# Autodesk Inventor assembly: arm_fin1
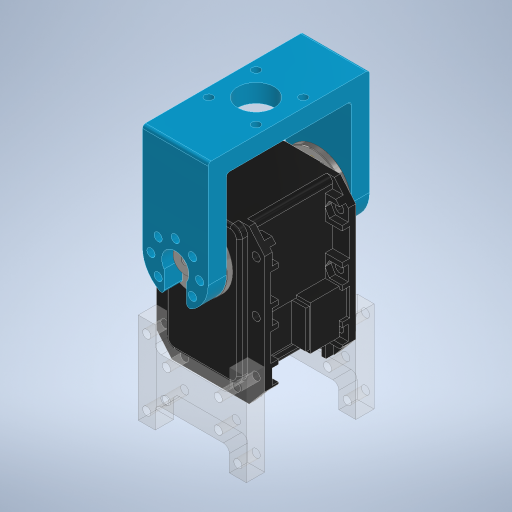
[picture p0: Inventor's stored thumbnail of the model, 512x512]
Saved by Autodesk Inventor 2024 (Build 280153000, 153)
## iProperties
Created: 2024-09-14
Part Number: arm_fin1
Document SubType Name: Assembly
Designer: jmha0
Author: jmha0
## Documents named in this file (6)
- C:\Users\jmha0\OneDrive\바탕 화면\19th_intern_hjm_fight_robot\Upper_Body\arm\arm_fin1.iam
- C:\Users\jmha0\OneDrive\바탕 화면\19th_intern_hjm_fight_robot\Upper_Body\arm\3D_upper_to_arm1.ipt
- C:\Users\jmha0\OneDrive\바탕 화면\19th_intern_hjm_fight_robot\hardware\ROBOTIS(Inventor 2024 ver.)\다이나믹셀\MX-28T_R+idle.ipt.iam
- C:\Users\jmha0\OneDrive\바탕 화면\19th_intern_hjm_fight_robot\hardware\ROBOTIS(Inventor 2024 ver.)\혼\28Horn.ipt
- C:\Users\jmha0\OneDrive\바탕 화면\19th_intern_hjm_fight_robot\Upper_Body\arm\frame_arm_to_hand1.ipt
- MX-28T_R+idle.ipt
## Components (5 placed, 4 different names)
1. 3D_upper_to_arm1:1 — 삽입:2, 삽입:3, 삽입:4, 삽입:5, 삽입:6, 삽입:7
2. MX-28T_R+idle.ipt:1 [sub-assembly] — 삽입:1, 삽입:5, 삽입:6, 삽입:7, 삽입:8, 삽입:9, 삽입:10, 삽입:11, 삽입:12, 삽입:13
3. 28Horn:1 — 삽입:1, 삽입:2, 삽입:3, 삽입:4
4. frame_arm_to_hand1:1 — 삽입:11, 삽입:12, 삽입:13
5. frame_arm_to_hand1:2 — 삽입:8, 삽입:9, 삽입:10
## Relationships (13: Insert 13)
- 삽입:1 [Insert] (0.1 mm): MX-28T_R+idle.ipt:1 ↔ 28Horn:1
- 삽입:2 [Insert]: 3D_upper_to_arm1:1 ↔ 28Horn:1
- 삽입:3 [Insert]: 3D_upper_to_arm1:1 ↔ 28Horn:1
- 삽입:4 [Insert]: 3D_upper_to_arm1:1 ↔ 28Horn:1
- 삽입:5 [Insert]: 3D_upper_to_arm1:1 ↔ MX-28T_R+idle.ipt:1
- 삽입:6 [Insert]: 3D_upper_to_arm1:1 ↔ MX-28T_R+idle.ipt:1
- 삽입:7 [Insert]: 3D_upper_to_arm1:1 ↔ MX-28T_R+idle.ipt:1
- 삽입:8 [Insert]: MX-28T_R+idle.ipt:1 ↔ frame_arm_to_hand1:2
- 삽입:9 [Insert]: MX-28T_R+idle.ipt:1 ↔ frame_arm_to_hand1:2
- 삽입:10 [Insert]: MX-28T_R+idle.ipt:1 ↔ frame_arm_to_hand1:2
- 삽입:11 [Insert]: MX-28T_R+idle.ipt:1 ↔ frame_arm_to_hand1:1
- 삽입:12 [Insert]: MX-28T_R+idle.ipt:1 ↔ frame_arm_to_hand1:1
- 삽입:13 [Insert]: MX-28T_R+idle.ipt:1 ↔ frame_arm_to_hand1:1
